# Autodesk Inventor assembly: nmt_pdu_assembly
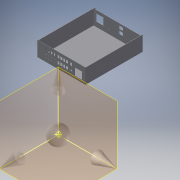
[picture p0: Inventor's stored thumbnail of the model, 180x180]
Saved by Autodesk Inventor 2017 (Build 210142000, 142)
## iProperties
Created: 2017-11-16
Part Number: nmt_pdu_assembly
Document SubType Name: Assembly
Designer: Zara
Author: Zara
## Documents named in this file (6)
- C:\Users\Zara\Documents\hera-cad\Node\NMT_PDU_merge\nmt_pdu_assembly.iam
- C:\Users\Zara\Documents\hera-cad\Node\NMT_PDU_merge\PDU_NMT_bottom.ipt
- C:\Users\Zara\Documents\hera-cad\Node\NMT_PDU_merge\PDU_NMT_sidepanel_right_20.ipt
- C:\Users\Zara\Documents\hera-cad\Node\NMT_PDU_merge\PDU_NMT_sidepanel_left_20.ipt
- C:\Users\Zara\Documents\hera-cad\Node\NMT_PDU_merge\PDU_chassis_back_merge.ipt
- C:\Users\Zara\Documents\hera-cad\Node\NMT_PDU_merge\PDU_NMT_front.ipt
## Components (5 placed, 5 different names)
1. PDU_NMT_bottom:1 — Flush:1, Mate:1, Mate:2, Flush:2, Flush:3, Mate:3, Mate:4, Flush:4
2. PDU_NMT_sidepanel_right_20:1 — Mate:2, Flush:2, Mate:7, Mate:8
3. PDU_NMT_sidepanel_left_20:1 — Mate:4, Flush:4, Mate:6
4. PDU_chassis_back_merge:1 — Flush:3, Mate:3
5. PDU_NMT_front:1 — Flush:1, Mate:1, Mate:6, Mate:7, Mate:8
## Relationships (11: Mate 7, Flush 4)
- Flush:1: PDU_NMT_bottom:1 ↔ PDU_NMT_front:1
- Mate:1: PDU_NMT_bottom:1 ↔ PDU_NMT_front:1
- Mate:2: PDU_NMT_bottom:1 ↔ PDU_NMT_sidepanel_right_20:1
- Flush:2: PDU_NMT_bottom:1 ↔ PDU_NMT_sidepanel_right_20:1
- Flush:3: PDU_NMT_bottom:1 ↔ PDU_chassis_back_merge:1
- Mate:3: PDU_NMT_bottom:1 ↔ PDU_chassis_back_merge:1
- Mate:4: PDU_NMT_bottom:1 ↔ PDU_NMT_sidepanel_left_20:1
- Flush:4: PDU_NMT_bottom:1 ↔ PDU_NMT_sidepanel_left_20:1
- Mate:6: PDU_NMT_sidepanel_left_20:1 ↔ PDU_NMT_front:1
- Mate:7: PDU_NMT_sidepanel_right_20:1 ↔ PDU_NMT_front:1
- Mate:8: PDU_NMT_sidepanel_right_20:1 ↔ PDU_NMT_front:1
